# Autodesk Inventor assembly: plasma-box-to-cathode-box-adapter
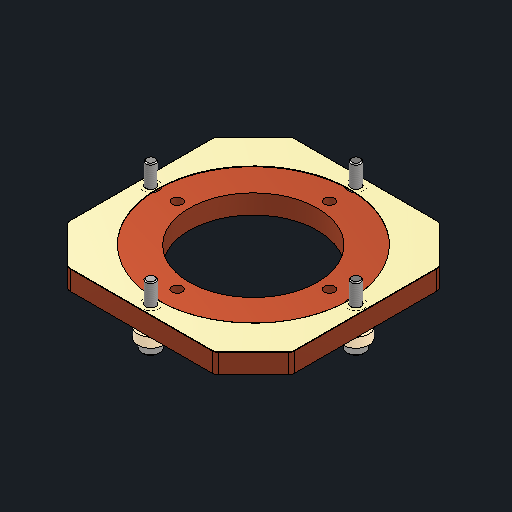
[picture p0: Inventor's stored thumbnail of the model, 512x512]
Saved by Autodesk Inventor 2026 (Build 300175050, 175E)
## iProperties
Created: 2024-06-26
Part Number: plasma-box-to-cathode-box-adapter
Document SubType Name: Assembly
Designer: kuzmin
Author: kuzmin
## Documents named in this file (5)
- C:\Users\queez\Dropbox\Drawings\PIHTI\Plasma Vessel\Plasma-Box\plasma-box-to-cathode-box-adapter.iam
- C:\Users\queez\Dropbox\Drawings\PIHTI\ContentCenter\Ceramics\ceramic_bushing_M3.ipt
- C:\Users\queez\Dropbox\Drawings\PIHTI\Plasma Vessel\Plasma-Box\plasma-box-spacer-6mm.ipt
- C:\Users\queez\Dropbox\Drawings\PIHTI\ContentCenter\Fastners\M3x16-SHCS.ipt
- C:\Users\queez\Dropbox\Drawings\PIHTI\Plasma Vessel\Plasma-Box\plasma-box-mica.ipt
## Components (10 placed, 4 different names)
1. ceramic_bushing_M3:1
2. plasma-box-spacer-6mm:1 — Rigid:6
3. ceramic_bushing_M3:2
4. ceramic_bushing_M3:3
5. ceramic_bushing_M3:4
6. plasma-box-mica:1 — Rigid:6
7. SS ISO 4762 M3 x 16:2
8. SS ISO 4762 M3 x 16:1
9. SS ISO 4762 M3 x 16:3
10. SS ISO 4762 M3 x 16:4
## Relationships (9: WeldJoint 6, RevoluteJoint 3)
- [WeldJoint]: ceramic_bushing_M3:1 ↔ SS ISO 4762 M3 x 16:1
- [WeldJoint]: ceramic_bushing_M3:2 ↔ SS ISO 4762 M3 x 16:2
- [WeldJoint]: ceramic_bushing_M3:3 ↔ SS ISO 4762 M3 x 16:3
- [WeldJoint]: ceramic_bushing_M3:4 ↔ SS ISO 4762 M3 x 16:4
- [WeldJoint]: plasma-box-spacer-6mm:1 ↔ ceramic_bushing_M3:2
- [RevoluteJoint]: plasma-box-spacer-6mm:1 ↔ ceramic_bushing_M3:3
- [RevoluteJoint]: plasma-box-spacer-6mm:1 ↔ ceramic_bushing_M3:4
- [RevoluteJoint]: ceramic_bushing_M3:1 ↔ plasma-box-spacer-6mm:1
- Rigid:6 [WeldJoint]: plasma-box-spacer-6mm:1 ↔ plasma-box-mica:1
## Named parameters: d112_d111 = 0 mm, d113_d111 = 0 mm, d114_d111 = 0 mm
